# Autodesk Inventor assembly: Pedal Assembly
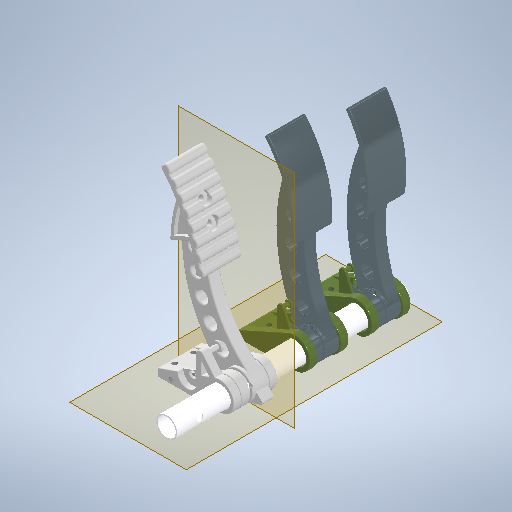
[picture p0: Inventor's stored thumbnail of the model, 512x512]
Saved by Autodesk Inventor 2025.2 (Build 292293000, 293)
## iProperties
Created: 2025-02-08
Part Number: Pedal Assembly
Document SubType Name: Assembly
Designer: eason
Author: eason
## Documents named in this file (9)
- C:\Users\eason\Desktop\Code\Unojoy-Simulator-Rig\CAD\Pedals\Pedal Assembly.iam
- C:\Users\eason\Desktop\Code\Unojoy-Simulator-Rig\CAD\Pedals\Steering PVC.ipt
- C:\Users\eason\Desktop\Code\Unojoy-Simulator-Rig\CAD\Pedals\Pedal Support.ipt
- C:\Users\eason\Desktop\Code\Unojoy-Simulator-Rig\CAD\Pedals\Pedal.ipt
- C:\Users\eason\Desktop\Code\Unojoy-Simulator-Rig\CAD\Pedals\Pedal 1.ipt
- C:\Users\eason\Desktop\Code\Unojoy-Simulator-Rig\CAD\Pedals\Pedal 2.ipt
- C:\Users\eason\Desktop\Code\Unojoy-Simulator-Rig\CAD\Pedals\Pedal Support 1.ipt
- C:\Users\eason\Desktop\Code\Unojoy-Simulator-Rig\CAD\Pedals\Pedal Support L.ipt
- C:\Users\eason\Desktop\Code\Unojoy-Simulator-Rig\CAD\Pedals\Pedal Support R.ipt
## Components (10 placed, 8 different names)
1. Steering PVC:1 — Cylindrical:1, Cylindrical:2, Cylindrical:4, Cylindrical:5, Cylindrical:6, Cylindrical:9
2. Pedal Support:1 — Mate:1, Cylindrical:1, Mate:4, Mate:7
3. Pedal:1 — Cylindrical:4, Mate:4
4. Pedal Support:2 — Mate:2, Cylindrical:2, Mate:5, Mate:7
5. Pedal:2 — Cylindrical:5, Mate:5
6. Pedal 1:1 — Cylindrical:6, Cylindrical:7, Cylindrical:8, Mate:10, Mate:11
7. Pedal 2:1 — Cylindrical:7, Cylindrical:8, Mate:10
8. Pedal Support 1:1 — Angle:1, Angle:2, Insert:1, Insert:2, Insert:3, Insert:4
9. Pedal Support L:1 — Cylindrical:9, Insert:2, Insert:3
10. Pedal Support R:1 — Insert:1, Insert:4, Mate:11, Mate:12
## Relationships (22: Mate 8, CylindricalJoint 8, Insert 4, Angle 2)
- Mate:1: Pedal Support:1
- Mate:2: Pedal Support:2
- Cylindrical:1: Steering PVC:1 ↔ Pedal Support:1
- Cylindrical:2: Steering PVC:1 ↔ Pedal Support:2
- Cylindrical:4: Steering PVC:1 ↔ Pedal:1
- Mate:4: Pedal Support:1 ↔ Pedal:1
- Cylindrical:5: Steering PVC:1 ↔ Pedal:2
- Mate:5: Pedal Support:2 ↔ Pedal:2
- Mate:7 (30 mm): Pedal Support:1 ↔ Pedal Support:2
- Cylindrical:6: Steering PVC:1 ↔ Pedal 1:1
- Cylindrical:7: Pedal 1:1 ↔ Pedal 2:1
- Cylindrical:8: Pedal 1:1 ↔ Pedal 2:1
- Mate:10: Pedal 1:1 ↔ Pedal 2:1
- Angle:1 (180 deg): Pedal Support 1:1
- Angle:2 (180 deg): Pedal Support 1:1
- Cylindrical:9: Steering PVC:1 ↔ Pedal Support L:1
- Insert:1: Pedal Support 1:1 ↔ Pedal Support R:1
- Insert:2: Pedal Support 1:1 ↔ Pedal Support L:1
- Insert:3: Pedal Support 1:1 ↔ Pedal Support L:1
- Insert:4: Pedal Support 1:1 ↔ Pedal Support R:1
- Mate:11 (0.2 mm): Pedal 1:1 ↔ Pedal Support R:1
- Mate:12: Pedal Support R:1
